# Autodesk Inventor assembly: fullCube
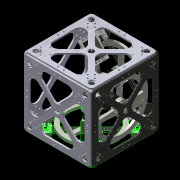
[picture p0: Inventor's stored thumbnail of the model, 180x180]
Saved by Autodesk Inventor 2018 (Build 220112000, 112)
## iProperties
Created: 2019-10-03
Part Number: fullCube
Document SubType Name: Assembly
Designer: anirudh
Author: anirudh
## Documents named in this file (4)
- C:\Users\anirudh\Documents\MARS Fund\Cubli\fullCube.iam
- C:\Users\anirudh\Documents\MARS Fund\Cubli\CAD Files\CubliAssembly.iam
- C:\Users\anirudh\Documents\MARS Fund\Cubli\CAD Files\CubliAssembly2.iam
- C:\Users\anirudh\Documents\MARS Fund\Cubli\CAD Files\SidePanel.ipt
## Components (6 placed, 3 different names)
1. CubliAssembly:1 [sub-assembly] — Flush:1, Mate:1, Flush:2, Mate:3, Mate:4, Mate:5, Mate:7, Mate:13
2. CubliAssembly:3 [sub-assembly] — Flush:1, Mate:1, Flush:2, Mate:2, Mate:6, Mate:8
3. CubliAssembly2:1 [sub-assembly] — Mate:2, Mate:3, Mate:4, Mate:9, Mate:12
4. SidePanel:1 — Mate:11, Mate:12, Mate:13
5. SidePanel:2 — Mate:8, Mate:9, Mate:10
6. SidePanel:3 — Mate:5, Mate:6, Mate:7, Mate:10, Mate:11
## Relationships (15: Mate 13, Flush 2)
- Flush:1 (3.5052 mm): CubliAssembly:1 ↔ CubliAssembly:3
- Mate:1: CubliAssembly:1 ↔ CubliAssembly:3
- Flush:2: CubliAssembly:1 ↔ CubliAssembly:3
- Mate:2: CubliAssembly:3 ↔ CubliAssembly2:1
- Mate:3: CubliAssembly:1 ↔ CubliAssembly2:1
- Mate:4: CubliAssembly:1 ↔ CubliAssembly2:1
- Mate:5: CubliAssembly:1 ↔ SidePanel:3
- Mate:6: CubliAssembly:3 ↔ SidePanel:3
- Mate:7: CubliAssembly:1 ↔ SidePanel:3
- Mate:8: CubliAssembly:3 ↔ SidePanel:2
- Mate:9: CubliAssembly2:1 ↔ SidePanel:2
- Mate:10: SidePanel:2 ↔ SidePanel:3
- Mate:11: SidePanel:1 ↔ SidePanel:3
- Mate:12: CubliAssembly2:1 ↔ SidePanel:1
- Mate:13: CubliAssembly:1 ↔ SidePanel:1
